# Autodesk Inventor assembly: x_carryage
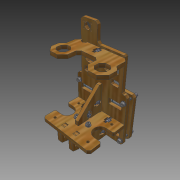
[picture p0: Inventor's stored thumbnail of the model, 180x180]
Saved by Autodesk Inventor 2014 (Build 180170000, 170)
## iProperties
Created: 2014-04-05
Part Number: x_carryage
Document SubType Name: Assembly
Designer: buben
Author: buben
## Documents named in this file (13)
- C:\Users\buben\Documents\GitHub\bacon\inventor files\assemblies\x_carryage.iam
- C:\Users\buben\Documents\GitHub\bacon\inventor files\printer parts\x_carryage_front.ipt
- C:\Users\buben\Documents\GitHub\bacon\inventor files\3rd party components\linear_bearing_8\Imported Components\LU8MM\LU8MM.iam
- C:\Users\buben\Documents\GitHub\bacon\inventor files\printer parts\x_carryage_back.ipt
- C:\Users\buben\Documents\GitHub\bacon\inventor files\printer parts\x_carryage_brace_bottom.ipt
- C:\Users\buben\Documents\GitHub\bacon\inventor files\printer parts\x_carryage_extruder_mount.ipt
- C:\Users\buben\Documents\GitHub\bacon\inventor files\printer parts\x_carryage_brace_top.ipt
- C:\Users\buben\Documents\GitHub\bacon\inventor files\utils\washer_m4.ipt
- C:\Users\buben\Documents\Inventor\Content Center Files\R2014\en-US\ISO 4762(2)\ISO 4762 - M4 x 30ISO.ipt
- C:\Users\buben\Documents\Inventor\Content Center Files\R2014\en-US\ISO 4762(2)\ISO 4762 - M4 x 20ISO.ipt
- C:\Users\buben\Documents\Inventor\Content Center Files\R2014\en-US\ISO 4762(2)\ISO 4762 - M4 x 35ISO.ipt
- C:\Users\buben\Documents\Inventor\Content Center Files\R2014\en-US\ISO 7040\ISO 7040 - M4.ipt
- C:\Users\buben\Documents\GitHub\bacon\inventor files\printer parts\filament_guide.ipt
## Components (64 placed, 12 different names)
1. x_carryage_front:1 — Mate:1, Mate:2, Flush:1, Mate:3, Mate:4, Mate:5, Mate:6, Mate:7, Mate:8, Mate:11, Mate:12, Flush:2, Flush:3, Mate:14, Mate:15, Flush:4, Flush:5, Mate:17, Flush:6, Mate:21, Mate:33, Mate:34, Mate:35, Mate:36, Mate:37, Mate:38, Mate:39, Mate:40, Mate:95, Mate:96, Mate:97, Mate:98, Mate:99
2. LU8MM:1 [sub-assembly] — Mate:3, Mate:4, Mate:5, Mate:9, Mate:13
3. LU8MM:2 [sub-assembly] — Mate:6, Mate:7, Mate:8, Mate:10
4. LU8MM:3 [sub-assembly] — Mate:9, Mate:12
5. LU8MM:4 [sub-assembly] — Mate:10, Mate:11
6. x_carryage_back:1 — Flush:2, Flush:3, Mate:13, Mate:23, Mate:24, Mate:25, Mate:26, Mate:27, Mate:28, Mate:29, Mate:30, Mate:31, Mate:32, Mate:47, Mate:49, Mate:51, Mate:53
7. x_carryage_brace_bottom:1 — Mate:14, Flush:4, Mate:16, Mate:18, Mate:57, Mate:67, Flush:7
8. x_carryage_brace_bottom:2 — Mate:15, Flush:5, Mate:19, Mate:59, Mate:69, Mate:104
9. x_carryage_extruder_mount:1 — Mate:16, Mate:17, Flush:6, Mate:18, Mate:19, Mate:20, Mate:22, Mate:41, Mate:42, Mate:43, Mate:44, Mate:45, Mate:46, Mate:63, Mate:65
10. x_carryage_brace_top:1 — Mate:20, Mate:21, Mate:22, Mate:55, Mate:61
11. CSN 02 1702 B B 4,3:1 — Mate:47, Mate:48, Mate:83
12. CSN 02 1702 B B 4,3:2 — Mate:45, Mate:46, Insert:7
13. CSN 02 1702 B B 4,3:3 — Mate:39, Mate:40, Insert:3
14. CSN 02 1702 B B 4,3:4 — Mate:57, Mate:58, Mate:91
15. CSN 02 1702 B B 4,3:5 — Mate:55, Mate:56, Mate:71
16. CSN 02 1702 B B 4,3:6 — Mate:41, Mate:42, Insert:6
17. CSN 02 1702 B B 4,3:7 — Mate:37, Mate:38, Insert:1
18. CSN 02 1702 B B 4,3:8 — Mate:43, Mate:44, Insert:5
19. CSN 02 1702 B B 4,3:9 — Mate:49, Mate:50, Mate:87
20. CSN 02 1702 B B 4,3:10 — Mate:59, Mate:60, Mate:93
21. CSN 02 1702 B B 4,3:11 — Mate:53, Mate:54, Mate:85
22. CSN 02 1702 B B 4,3:12 — Mate:61, Mate:62, Mate:73
23. CSN 02 1702 B B 4,3:13 — Mate:51, Mate:52, Mate:89
24. CSN 02 1702 B B 4,3:14 — Mate:29, Mate:30, Insert:12
25. CSN 02 1702 B B 4,3:15 — Mate:23, Mate:24, Insert:8
26. CSN 02 1702 B B 4,3:16 — Mate:25, Mate:26, Insert:10
27. CSN 02 1702 B B 4,3:17 — Mate:27, Mate:28, Insert:9
28. CSN 02 1702 B B 4,3:18 — Mate:31, Mate:32, Insert:11
29. CSN 02 1702 B B 4,3:19 — Mate:33, Mate:34, Insert:2
30. CSN 02 1702 B B 4,3:20 — Mate:35, Mate:36, Insert:4
31. ISO 4762 M4 x 30:1 — Insert:1, Mate:52, Mate:90
32. ISO 4762 M4 x 30:2 — Insert:2, Mate:50, Mate:88
33. ISO 4762 M4 x 30:3 — Insert:3, Mate:54, Mate:86
34. ISO 4762 M4 x 30:4 — Insert:4, Mate:48, Mate:84
35. ISO 4762 M4 x 20:1 — Insert:5, Mate:60, Mate:94
36. ISO 4762 M4 x 20:2 — Insert:6, Mate:58, Mate:92
37. ISO 4762 M4 x 20:3 — Insert:7, Mate:56, Mate:72
38. ISO 4762 M4 x 35:1 — Insert:8, Mate:62, Mate:74
39. ISO 4762 M4 x 35:2 — Insert:9, Mate:66, Mate:78
40. ISO 4762 M4 x 35:3 — Insert:10, Mate:64, Mate:76
41. ISO 4762 M4 x 35:4 — Insert:11, Mate:70, Mate:82
42. ISO 4762 M4 x 35:5 — Insert:12, Mate:68, Mate:80
43. CSN 02 1702 B B 4,3:21 — Mate:63, Mate:64, Mate:75
44. CSN 02 1702 B B 4,3:22 — Mate:67, Mate:68, Mate:79
45. CSN 02 1702 B B 4,3:23 — Mate:69, Mate:70, Mate:81
46. CSN 02 1702 B B 4,3:24 — Mate:65, Mate:66, Mate:77
47. DIN EN ISO 7040 M4:1 — Mate:71, Mate:72
48. DIN EN ISO 7040 M4:2 — Mate:81, Mate:82
49. DIN EN ISO 7040 M4:3 — Mate:85, Mate:86
50. DIN EN ISO 7040 M4:4 — Mate:87, Mate:88
51. DIN EN ISO 7040 M4:5 — Mate:83, Mate:84
52. DIN EN ISO 7040 M4:6 — Mate:79, Mate:80
53. DIN EN ISO 7040 M4:7 — Mate:77, Mate:78
54. DIN EN ISO 7040 M4:8 — Mate:75, Mate:76
55. DIN EN ISO 7040 M4:9 — Mate:73, Mate:74
56. DIN EN ISO 7040 M4:10 — Mate:89, Mate:90
57. DIN EN ISO 7040 M4:11 — Mate:93, Mate:94
58. DIN EN ISO 7040 M4:12 — Mate:91, Mate:92
59. filament_guide:1 — Mate:95, Mate:96, Mate:97, Mate:100
60. CSN 02 1702 B B 4,3:25 — Mate:98, Mate:99, Insert:13
61. CSN 02 1702 B B 4,3:26 — Mate:100, Mate:101, Mate:102
62. ISO 4762 M4 x 20:4 — Insert:13, Mate:101, Mate:103
63. DIN EN ISO 7040 M4:13 — Mate:102, Mate:103
64. LU8MM:5 [sub-assembly] — Mate:104, Flush:7
## Relationships (124: Mate 104, Insert 13, Flush 7)
- Mate:1: x_carryage_front:1
- Mate:2: x_carryage_front:1
- Flush:1: x_carryage_front:1
- Mate:3 (7.5 mm): x_carryage_front:1 ↔ LU8MM:1
- Mate:4 (7.5 mm): x_carryage_front:1 ↔ LU8MM:1
- Mate:5 (0.5 mm): x_carryage_front:1 ↔ LU8MM:1
- Mate:6 (7.5 mm): x_carryage_front:1 ↔ LU8MM:2
- Mate:7 (7.5 mm): x_carryage_front:1 ↔ LU8MM:2
- Mate:8 (0.5 mm): x_carryage_front:1 ↔ LU8MM:2
- Mate:9: LU8MM:1 ↔ LU8MM:3
- Mate:10: LU8MM:2 ↔ LU8MM:4
- Mate:11 (0.5 mm): x_carryage_front:1 ↔ LU8MM:4
- Mate:12 (0.5 mm): x_carryage_front:1 ↔ LU8MM:3
- Flush:2: x_carryage_front:1 ↔ x_carryage_back:1
- Flush:3: x_carryage_front:1 ↔ x_carryage_back:1
- Mate:13 (7.5 mm): LU8MM:1 ↔ x_carryage_back:1
- Mate:14: x_carryage_front:1 ↔ x_carryage_brace_bottom:1
- Mate:15: x_carryage_front:1 ↔ x_carryage_brace_bottom:2
- Flush:4: x_carryage_front:1 ↔ x_carryage_brace_bottom:1
- Flush:5: x_carryage_front:1 ↔ x_carryage_brace_bottom:2
- Mate:16: x_carryage_brace_bottom:1 ↔ x_carryage_extruder_mount:1
- Mate:17: x_carryage_front:1 ↔ x_carryage_extruder_mount:1
- Flush:6: x_carryage_front:1 ↔ x_carryage_extruder_mount:1
- Mate:18: x_carryage_brace_bottom:1 ↔ x_carryage_extruder_mount:1
- Mate:19: x_carryage_brace_bottom:2 ↔ x_carryage_extruder_mount:1
- Mate:20: x_carryage_extruder_mount:1 ↔ x_carryage_brace_top:1
- Mate:21: x_carryage_front:1 ↔ x_carryage_brace_top:1
- Mate:22: x_carryage_extruder_mount:1 ↔ x_carryage_brace_top:1
- Mate:23: x_carryage_back:1 ↔ CSN 02 1702 B B 4,3:15
- Mate:24: x_carryage_back:1 ↔ CSN 02 1702 B B 4,3:15
- Mate:25: x_carryage_back:1 ↔ CSN 02 1702 B B 4,3:16
- Mate:26: x_carryage_back:1 ↔ CSN 02 1702 B B 4,3:16
- Mate:27: x_carryage_back:1 ↔ CSN 02 1702 B B 4,3:17
- Mate:28: x_carryage_back:1 ↔ CSN 02 1702 B B 4,3:17
- Mate:29: x_carryage_back:1 ↔ CSN 02 1702 B B 4,3:14
- Mate:30: x_carryage_back:1 ↔ CSN 02 1702 B B 4,3:14
- Mate:31: x_carryage_back:1 ↔ CSN 02 1702 B B 4,3:18
- Mate:32: x_carryage_back:1 ↔ CSN 02 1702 B B 4,3:18
- Mate:33: x_carryage_front:1 ↔ CSN 02 1702 B B 4,3:19
- Mate:34: x_carryage_front:1 ↔ CSN 02 1702 B B 4,3:19
- Mate:35: x_carryage_front:1 ↔ CSN 02 1702 B B 4,3:20
- Mate:36: x_carryage_front:1 ↔ CSN 02 1702 B B 4,3:20
- Mate:37: x_carryage_front:1 ↔ CSN 02 1702 B B 4,3:7
- Mate:38: x_carryage_front:1 ↔ CSN 02 1702 B B 4,3:7
- Mate:39: x_carryage_front:1 ↔ CSN 02 1702 B B 4,3:3
- Mate:40: x_carryage_front:1 ↔ CSN 02 1702 B B 4,3:3
- Mate:41: x_carryage_extruder_mount:1 ↔ CSN 02 1702 B B 4,3:6
- Mate:42: x_carryage_extruder_mount:1 ↔ CSN 02 1702 B B 4,3:6
- Mate:43: x_carryage_extruder_mount:1 ↔ CSN 02 1702 B B 4,3:8
- Mate:44: x_carryage_extruder_mount:1 ↔ CSN 02 1702 B B 4,3:8
- Mate:45: x_carryage_extruder_mount:1 ↔ CSN 02 1702 B B 4,3:2
- Mate:46: x_carryage_extruder_mount:1 ↔ CSN 02 1702 B B 4,3:2
- Insert:1: CSN 02 1702 B B 4,3:7 ↔ ISO 4762 M4 x 30:1
- Insert:2: CSN 02 1702 B B 4,3:19 ↔ ISO 4762 M4 x 30:2
- Insert:3: CSN 02 1702 B B 4,3:3 ↔ ISO 4762 M4 x 30:3
- Insert:4: CSN 02 1702 B B 4,3:20 ↔ ISO 4762 M4 x 30:4
- Mate:47: x_carryage_back:1 ↔ CSN 02 1702 B B 4,3:1
- Mate:48: CSN 02 1702 B B 4,3:1 ↔ ISO 4762 M4 x 30:4
- Mate:49: x_carryage_back:1 ↔ CSN 02 1702 B B 4,3:9
- Mate:50: CSN 02 1702 B B 4,3:9 ↔ ISO 4762 M4 x 30:2
- Mate:51: x_carryage_back:1 ↔ CSN 02 1702 B B 4,3:13
- Mate:52: CSN 02 1702 B B 4,3:13 ↔ ISO 4762 M4 x 30:1
- Mate:53: x_carryage_back:1 ↔ CSN 02 1702 B B 4,3:11
- Mate:54: CSN 02 1702 B B 4,3:11 ↔ ISO 4762 M4 x 30:3
- Insert:5: CSN 02 1702 B B 4,3:8 ↔ ISO 4762 M4 x 20:1
- Insert:6: CSN 02 1702 B B 4,3:6 ↔ ISO 4762 M4 x 20:2
- Insert:7: CSN 02 1702 B B 4,3:2 ↔ ISO 4762 M4 x 20:3
- Mate:55: x_carryage_brace_top:1 ↔ CSN 02 1702 B B 4,3:5
- Mate:56: CSN 02 1702 B B 4,3:5 ↔ ISO 4762 M4 x 20:3
- Mate:57: x_carryage_brace_bottom:1 ↔ CSN 02 1702 B B 4,3:4
- Mate:58: CSN 02 1702 B B 4,3:4 ↔ ISO 4762 M4 x 20:2
- Mate:59: x_carryage_brace_bottom:2 ↔ CSN 02 1702 B B 4,3:10
- Mate:60: CSN 02 1702 B B 4,3:10 ↔ ISO 4762 M4 x 20:1
- Insert:8: CSN 02 1702 B B 4,3:15 ↔ ISO 4762 M4 x 35:1
- Insert:9: CSN 02 1702 B B 4,3:17 ↔ ISO 4762 M4 x 35:2
- Insert:10: CSN 02 1702 B B 4,3:16 ↔ ISO 4762 M4 x 35:3
- Insert:11: CSN 02 1702 B B 4,3:18 ↔ ISO 4762 M4 x 35:4
- Insert:12: CSN 02 1702 B B 4,3:14 ↔ ISO 4762 M4 x 35:5
- Mate:61: x_carryage_brace_top:1 ↔ CSN 02 1702 B B 4,3:12
- Mate:62: CSN 02 1702 B B 4,3:12 ↔ ISO 4762 M4 x 35:1
- Mate:63: x_carryage_extruder_mount:1 ↔ CSN 02 1702 B B 4,3:21
- Mate:64: ISO 4762 M4 x 35:3 ↔ CSN 02 1702 B B 4,3:21
- Mate:65: x_carryage_extruder_mount:1 ↔ CSN 02 1702 B B 4,3:24
- Mate:66: ISO 4762 M4 x 35:2 ↔ CSN 02 1702 B B 4,3:24
- Mate:67: x_carryage_brace_bottom:1 ↔ CSN 02 1702 B B 4,3:22
- Mate:68: ISO 4762 M4 x 35:5 ↔ CSN 02 1702 B B 4,3:22
- Mate:69: x_carryage_brace_bottom:2 ↔ CSN 02 1702 B B 4,3:23
- Mate:70: ISO 4762 M4 x 35:4 ↔ CSN 02 1702 B B 4,3:23
- Mate:71: CSN 02 1702 B B 4,3:5 ↔ DIN EN ISO 7040 M4:1
- Mate:72: ISO 4762 M4 x 20:3 ↔ DIN EN ISO 7040 M4:1
- Mate:73: CSN 02 1702 B B 4,3:12 ↔ DIN EN ISO 7040 M4:9
- Mate:74: ISO 4762 M4 x 35:1 ↔ DIN EN ISO 7040 M4:9
- Mate:75: CSN 02 1702 B B 4,3:21 ↔ DIN EN ISO 7040 M4:8
- Mate:76: ISO 4762 M4 x 35:3 ↔ DIN EN ISO 7040 M4:8
- Mate:77: CSN 02 1702 B B 4,3:24 ↔ DIN EN ISO 7040 M4:7
- Mate:78: ISO 4762 M4 x 35:2 ↔ DIN EN ISO 7040 M4:7
- Mate:79: CSN 02 1702 B B 4,3:22 ↔ DIN EN ISO 7040 M4:6
- Mate:80: ISO 4762 M4 x 35:5 ↔ DIN EN ISO 7040 M4:6
- Mate:81: CSN 02 1702 B B 4,3:23 ↔ DIN EN ISO 7040 M4:2
- Mate:82: ISO 4762 M4 x 35:4 ↔ DIN EN ISO 7040 M4:2
- Mate:83: CSN 02 1702 B B 4,3:1 ↔ DIN EN ISO 7040 M4:5
- Mate:84: ISO 4762 M4 x 30:4 ↔ DIN EN ISO 7040 M4:5
- Mate:85: CSN 02 1702 B B 4,3:11 ↔ DIN EN ISO 7040 M4:3
- Mate:86: ISO 4762 M4 x 30:3 ↔ DIN EN ISO 7040 M4:3
- Mate:87: CSN 02 1702 B B 4,3:9 ↔ DIN EN ISO 7040 M4:4
- Mate:88: ISO 4762 M4 x 30:2 ↔ DIN EN ISO 7040 M4:4
- Mate:89: CSN 02 1702 B B 4,3:13 ↔ DIN EN ISO 7040 M4:10
- Mate:90: ISO 4762 M4 x 30:1 ↔ DIN EN ISO 7040 M4:10
- Mate:91: CSN 02 1702 B B 4,3:4 ↔ DIN EN ISO 7040 M4:12
- Mate:92: ISO 4762 M4 x 20:2 ↔ DIN EN ISO 7040 M4:12
- Mate:93: CSN 02 1702 B B 4,3:10 ↔ DIN EN ISO 7040 M4:11
- Mate:94: ISO 4762 M4 x 20:1 ↔ DIN EN ISO 7040 M4:11
- Mate:95: x_carryage_front:1 ↔ filament_guide:1
- Mate:96: x_carryage_front:1 ↔ filament_guide:1
- Mate:97: x_carryage_front:1 ↔ filament_guide:1
- Mate:98: x_carryage_front:1 ↔ CSN 02 1702 B B 4,3:25
- Mate:99: x_carryage_front:1 ↔ CSN 02 1702 B B 4,3:25
- Mate:100: filament_guide:1 ↔ CSN 02 1702 B B 4,3:26
- Insert:13: CSN 02 1702 B B 4,3:25 ↔ ISO 4762 M4 x 20:4
- Mate:101: CSN 02 1702 B B 4,3:26 ↔ ISO 4762 M4 x 20:4
- Mate:102: CSN 02 1702 B B 4,3:26 ↔ DIN EN ISO 7040 M4:13
- Mate:103: ISO 4762 M4 x 20:4 ↔ DIN EN ISO 7040 M4:13
- Mate:104: x_carryage_brace_bottom:2 ↔ LU8MM:5
- Flush:7 (3.75 mm): x_carryage_brace_bottom:1 ↔ LU8MM:5
